# Autodesk Inventor assembly: Mithril Cover
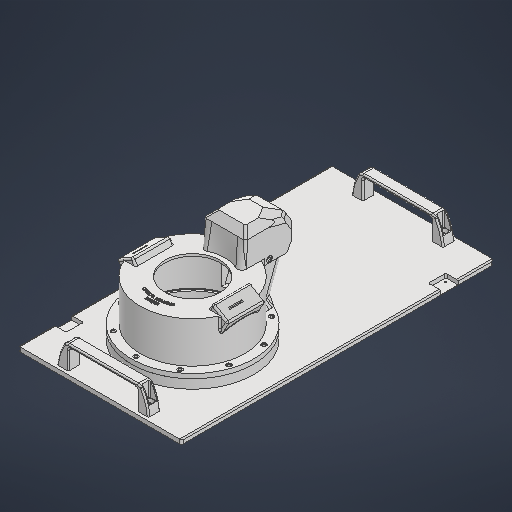
[picture p0: Inventor's stored thumbnail of the model, 512x512]
Saved by Autodesk Inventor 2026.2 (Build 302298000, 298)
## iProperties
Created: 2026-01-15
Part Number: Mithril Cover
Document SubType Name: Assembly
Designer: mumin
Author: mumin
## Documents named in this file (6)
- C:\GitHub\In-situ-monitoring-of-powder-bed-fusion-additive-manufacturing\system_development\Mithril\v0.4\Mithril Cover.iam
- C:\GitHub\In-situ-monitoring-of-powder-bed-fusion-additive-manufacturing\system_development\Mithril\v0.4\12mm Cover.ipt
- C:\GitHub\In-situ-monitoring-of-powder-bed-fusion-additive-manufacturing\system_development\Mithril\v0.4\Camera Cylinder Housing.ipt
- C:\GitHub\In-situ-monitoring-of-powder-bed-fusion-additive-manufacturing\system_development\Mithril\v0.4\SealedGlassRing.ipt
- C:\GitHub\In-situ-monitoring-of-powder-bed-fusion-additive-manufacturing\system_development\Mithril\v0.4\Handle.ipt
- C:\GitHub\In-situ-monitoring-of-powder-bed-fusion-additive-manufacturing\system_development\Mithril\v0.4\New Camera Lid.ipt
## Components (6 placed, 5 different names)
1. 12mm Cover:1 — Insert:1, Insert:3, Insert:4, Insert:5
2. Camera Cylinder Housing:1 — Insert:2, Mate:1, Insert:6, Mate:2, Mate:3
3. SealedGlassRing:1 — Insert:1, Insert:2, Insert:5, Insert:6
4. Handle:1 — Insert:3
5. Handle:2 — Insert:4
6. New Camera Lid:1 — Mate:1, Mate:2, Mate:3
## Relationships (9: Insert 6, Mate 3)
- Insert:1: 12mm Cover:1 ↔ SealedGlassRing:1
- Insert:2: Camera Cylinder Housing:1 ↔ SealedGlassRing:1
- Insert:3: 12mm Cover:1 ↔ Handle:1
- Insert:4: 12mm Cover:1 ↔ Handle:2
- Mate:1: Camera Cylinder Housing:1 ↔ New Camera Lid:1
- Insert:5: 12mm Cover:1 ↔ SealedGlassRing:1
- Insert:6: Camera Cylinder Housing:1 ↔ SealedGlassRing:1
- Mate:2: Camera Cylinder Housing:1 ↔ New Camera Lid:1
- Mate:3: Camera Cylinder Housing:1 ↔ New Camera Lid:1
